# Autodesk Inventor assembly: DoubleCrossTestAsm
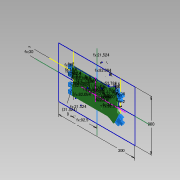
[picture p0: Inventor's stored thumbnail of the model, 180x180]
Saved by Autodesk Inventor 2021 (Build 250183000, 183)
## iProperties
Created: 2021-02-18
Part Number: DoubleCrossTestAsm
Document SubType Name: Assembly
Designer: kumagai
Author: kumagai
## Documents named in this file (5)
- X:\Develop\CAD\PlaRails\DoubleCross\DoubleCrossTestAsm.iam
- X:\Develop\CAD\PlaRails\DoubleCross\DoubleCrossRail.iam
- X:\Develop\CAD\PlaRails\DoubleCross\DoubleCrossBar.ipt
- X:\Develop\CAD\PlaRails\DoubleCross\DoubleCrossBar_MIR.ipt
- X:\Develop\CAD\PlaRails\DoubleCross\DoubleCrossBarPin.ipt
## Components (9 placed, 4 different names)
1. DoubleCrossRail:1 [sub-assembly] — メイト:1, メイト:2, メイト:3, メイト:4, メイト:5, メイト:6, メイト:7, メイト:8
2. DoubleCrossBar:1 — メイト:1, メイト:5, 回転:2
3. DoubleCrossBar_MIR:1 — メイト:3, メイト:8, 回転:3
4. DoubleCrossBar:2 — メイト:4, メイト:7, 回転:4
5. DoubleCrossBar_MIR:2 — メイト:2, メイト:6, 回転:1
6. DoubleCrossBarPin:1 — 回転:2
7. DoubleCrossBarPin:2 — 回転:1
8. DoubleCrossBarPin:3 — 回転:4
9. DoubleCrossBarPin:4 — 回転:3
## Relationships (12: Mate 8, RevoluteJoint 4)
- メイト:1 [Mate]: DoubleCrossRail:1 ↔ DoubleCrossBar:1
- メイト:2 [Mate]: DoubleCrossRail:1 ↔ DoubleCrossBar_MIR:2
- メイト:3 [Mate]: DoubleCrossRail:1 ↔ DoubleCrossBar_MIR:1
- メイト:4 [Mate]: DoubleCrossRail:1 ↔ DoubleCrossBar:2
- メイト:5 [Mate]: DoubleCrossRail:1 ↔ DoubleCrossBar:1
- メイト:6 [Mate]: DoubleCrossRail:1 ↔ DoubleCrossBar_MIR:2
- メイト:7 [Mate]: DoubleCrossRail:1 ↔ DoubleCrossBar:2
- メイト:8 [Mate]: DoubleCrossRail:1 ↔ DoubleCrossBar_MIR:1
- 回転:1 [RevoluteJoint]: DoubleCrossBar_MIR:2 ↔ DoubleCrossBarPin:2
- 回転:2 [RevoluteJoint]: DoubleCrossBar:1 ↔ DoubleCrossBarPin:1
- 回転:3 [RevoluteJoint]: DoubleCrossBar_MIR:1 ↔ DoubleCrossBarPin:4
- 回転:4 [RevoluteJoint]: DoubleCrossBar:2 ↔ DoubleCrossBarPin:3
